# Autodesk Inventor assembly: Assembly_Matchboxscope_injectionmolded_holo
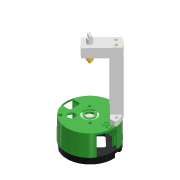
[picture p0: Inventor's stored thumbnail of the model, 180x180]
Saved by Autodesk Inventor 2022 (Build 260153000, 153)
## iProperties
Created: 2023-04-12
Part Number: Assembly_Matchboxscope_injectionmolded_holo
Document SubType Name: Assembly
Designer: diederichbenedict
Author: diederichbenedict
## Documents named in this file (8)
- C:\Users\diederichbenedict\Dropbox\Dokumente\Promotion\PROJECTS\Matchboxscope\INVENTOR\RELEASE\InjectionMolded\Assembly_Matchboxscope_injectionmolded_holo.iam
- C:\Users\diederichbenedict\Dropbox\Dokumente\Promotion\PROJECTS\Matchboxscope\INVENTOR\RELEASE\InjectionMolded\IM_Matchboxscope_base.ipt
- C:\Users\diederichbenedict\Dropbox\Dokumente\Promotion\PROJECTS\Matchboxscope\INVENTOR\RELEASE\InjectionMolded\IM_Matchboxscope_plate.ipt
- C:\Users\diederichbenedict\Dropbox\Dokumente\Promotion\PROJECTS\Matchboxscope\INVENTOR\RELEASE\InjectionMolded\Anglerfish_Cameraspacer.ipt
- C:\Users\diederichbenedict\Dropbox\Dokumente\Promotion\PROJECTS\Matchboxscope\INVENTOR\RELEASE\InjectionMolded\00_laserpointer_red.ipt
- C:\Users\diederichbenedict\Dropbox\Dokumente\Promotion\PROJECTS\Matchboxscope\INVENTOR\RELEASE\InjectionMolded\00_mk8_nozzle_0.4STEP.ipt
- C:\Users\diederichbenedict\Dropbox\Dokumente\Promotion\PROJECTS\Matchboxscope\INVENTOR\RELEASE\InjectionMolded\IM_Matchboxscope_Laserholder.ipt
- C:\Users\diederichbenedict\Dropbox\Dokumente\Promotion\PROJECTS\Matchboxscope\INVENTOR\RELEASE\InjectionMolded\IM_Matchboxscope_Laserholder_2.ipt
## Components (7 placed, 7 different names)
1. IM_Matchboxscope_base:1 — Passend:1, Passend:2, Fluchtend:1, Fluchtend:2
2. IM_Matchboxscope_plate:1
3. Anglerfish_Cameraspacer:1
4. 00_laserpointer_red:2 — Einfügen:3, Passend:1
5. 00_mk8_nozzle_0.4STEP:1 — Einfügen:3, Passend:2
6. IM_Matchboxscope_Laserholder:1 — Fluchtend:1, Fluchtend:2, Fluchtend:3
7. IM_Matchboxscope_Laserholder_2:1 — Fluchtend:3
## Relationships (8: Insert 3, Flush 3, Mate 2)
- [Insert]: IM_Matchboxscope_base:1 ↔ IM_Matchboxscope_plate:1
- [Insert]: IM_Matchboxscope_base:1 ↔ IM_Matchboxscope_plate:1
- Einfügen:3 [Insert] (2 mm): 00_laserpointer_red:2 ↔ 00_mk8_nozzle_0.4STEP:1
- Passend:1 [Mate]: IM_Matchboxscope_base:1 ↔ 00_laserpointer_red:2
- Passend:2 [Mate] (50 mm): IM_Matchboxscope_base:1 ↔ 00_mk8_nozzle_0.4STEP:1
- Fluchtend:1 [Flush]: IM_Matchboxscope_base:1 ↔ IM_Matchboxscope_Laserholder:1
- Fluchtend:2 [Flush]: IM_Matchboxscope_base:1 ↔ IM_Matchboxscope_Laserholder:1
- Fluchtend:3 [Flush]: IM_Matchboxscope_Laserholder:1 ↔ IM_Matchboxscope_Laserholder_2:1
